# Autodesk Inventor assembly: masbrobot2 1
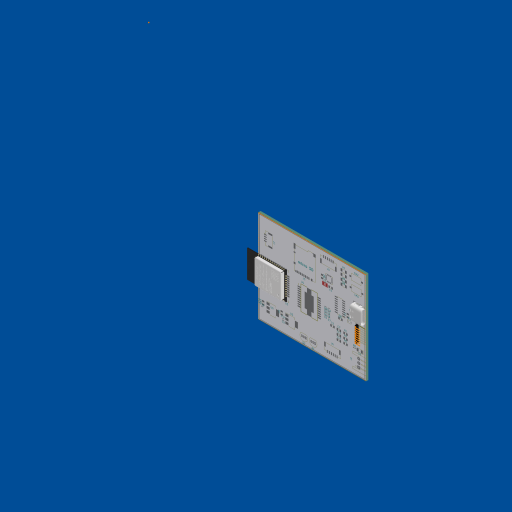
[picture p0: Inventor's stored thumbnail of the model, 512x512]
Saved by Autodesk Inventor 2023.1 (Build 271208000, 208)
## iProperties
Company: Kicad
Created: 2023-06-05
Part Number: masbrobot2 1
Description: KiCad electronic assembly
Document SubType Name: Assembly
Designer: nara atthama
Authority: Unknown
Sending System: KiCad to STEP converter
Preprocessor: Open CASCADE STEP processor 7.6
Title: masbrobot2.step
Author: Pcbnew
## Documents named in this file (5)
- C:\Users\naraa\OneDrive - Universitas Airlangga\Dokumen\kuliah\MATKUL\sem6\TopSus\masbrobot\model\masbrobot2.iam
- C:\Users\naraa\OneDrive - Universitas Airlangga\Dokumen\kuliah\MATKUL\sem6\TopSus\masbrobot\model\TYPE-C-31-M-12.iam
- C:\Users\naraa\OneDrive - Universitas Airlangga\Dokumen\kuliah\MATKUL\sem6\TopSus\masbrobot\model\masbrobot PCB.ipt
- C:\Users\naraa\OneDrive - Universitas Airlangga\Dokumen\kuliah\MATKUL\sem6\TopSus\masbrobot\model\pin-header-right-male-2-54mm-1-row-1.snapshot.1\Pin header right 1 row\PinHeader_8X1_right.ipt
- C:\Users\naraa\OneDrive - Universitas Airlangga\Dokumen\kuliah\MATKUL\sem6\TopSus\masbrobot\model\esp32-wroom-32d\ESP32-WROOM-32D.ipt
## Components (4 placed, 4 different names)
1. 2 [sub-assembly]
2. 3 — Mate:1, Flush:1, Mate:2, Flush:2
3. PinHeader_8X1_right:1 — Mate:1, Flush:1
4. ESP32-WROOM-32D:1 — Mate:2, Flush:2
## Relationships (4: Mate 2, Flush 2)
- Mate:1: 3 ↔ PinHeader_8X1_right:1
- Flush:1 (-4.7 mm): 3 ↔ PinHeader_8X1_right:1
- Mate:2: 3 ↔ ESP32-WROOM-32D:1
- Flush:2: 3 ↔ ESP32-WROOM-32D:1
